# Autodesk Inventor assembly: RadKomplet
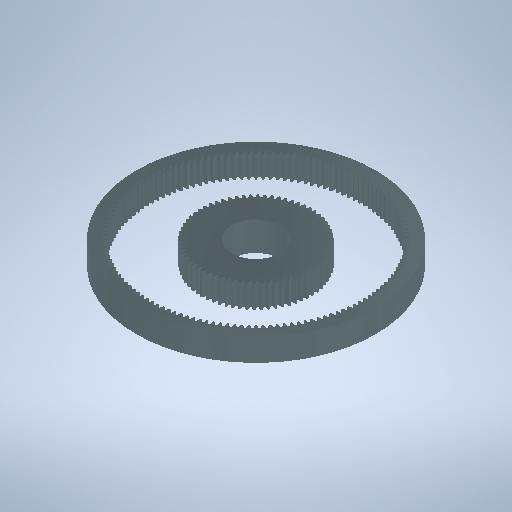
[picture p0: Inventor's stored thumbnail of the model, 512x512]
Saved by Autodesk Inventor 2025 (Build 290162010, 162A)
## iProperties
Created: 2024-07-15
Part Number: RadKomplet
Document SubType Name: Assembly
Designer: ffogue
Author: ffogue
## Documents named in this file (3)
- C:\Users\ffogue\OneDrive - MuM - OM\Dokumente\Inventor\Boxermotor\RadKomplet.iam
- C:\Users\ffogue\OneDrive - MuM - OM\Dokumente\Inventor\Boxermotor\PlanetenRad.ipt
- C:\Users\ffogue\OneDrive - MuM - OM\Dokumente\Inventor\Boxermotor\Stirnzahnrad12.ipt
## Components (2 placed, 1 different names)
1. Stirnzahnrad1:1 — Mate:1, Flush:1, Rotation:1, Mate:4
2. Stirnzahnrad1:2 — Mate:2, Flush:1, Angle:1, Rotation:1
## Relationships (7: Mate 4, Flush 1, Angle 1, RelateRotation 1)
- Mate:1: Stirnzahnrad1:1
- Mate:2: Stirnzahnrad1:2
- Mate:3
- Flush:1: Stirnzahnrad1:1 ↔ Stirnzahnrad1:2
- Angle:1 (0 deg): Stirnzahnrad1:2
- Rotation:1 [RelateRotation] (0.4783 ul): Stirnzahnrad1:1 ↔ Stirnzahnrad1:2
- Mate:4: Stirnzahnrad1:1
